# Autodesk Inventor assembly: PowerHub
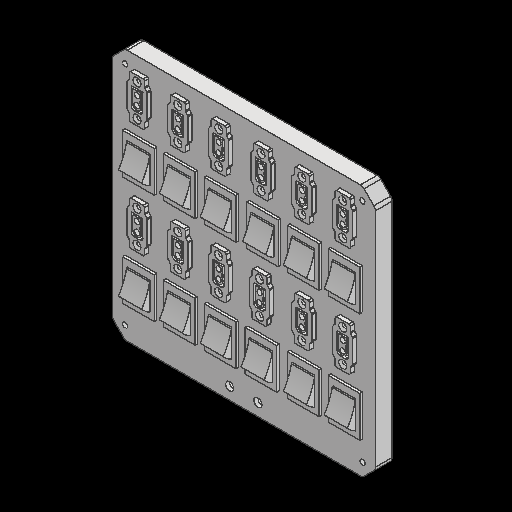
[picture p0: Inventor's stored thumbnail of the model, 512x512]
Saved by Autodesk Inventor 2025.2 (Build 292293000, 293)
## iProperties
Created: 2026-06-06
Part Number: PowerHub
Document SubType Name: Assembly
Designer: valer
Author: valer
## Documents named in this file (4)
- C:\Users\valer\Desktop\str1ker\cad\PowerHub.iam
- C:\Users\valer\Desktop\str1ker\cad\PowerHub.ipt
- C:\Users\valer\Desktop\str1ker\cad\external\XT60E-F.ipt
- C:\Users\valer\Desktop\str1ker\cad\external\IlluminatedSwitch12V10A.ipt
## Components (25 placed, 3 different names)
1. PowerHub:1 — Flush:2, Flush:3, Mate:1, Mate:2, Mate:3, Flush:5, Flush:6, Mate:16, Mate:17, Mate:18, Mate:19, Mate:20, Mate:21, Flush:35, Mate:22, Mate:23, Mate:24, Mate:26, Mate:27, Mate:32, Mate:33, Mate:34, Mate:36, Mate:37, Mate:39, Mate:40, Mate:42, Mate:43, Mate:44, Mate:45
2. XT60E-F:1 — Mate:2, Flush:4, Flush:5, Mate:4, Flush:6, Flush:30, Flush:36, Mate:28
3. IlluminatedSwitch12V10A:1 — Mate:3, Flush:4, Mate:4, Mate:25
4. XT60E-F:2 — Mate:16, Flush:30, Flush:31, Mate:28, Mate:29
5. IlluminatedSwitch12V10A:2 — Mate:17
6. XT60E-F:3 — Flush:31, Flush:32, Mate:22, Mate:29
7. IlluminatedSwitch12V10A:3 — Mate:18
8. XT60E-F:4 — Mate:19, Flush:32, Flush:33, Mate:31
9. IlluminatedSwitch12V10A:4 — Mate:34
10. XT60E-F:5 — Mate:20, Flush:33, Flush:34, Mate:30, Mate:31, Flush:43
11. IlluminatedSwitch12V10A:5 — Mate:33
12. XT60E-F:6 — Mate:21, Flush:34, Flush:35, Mate:30, Flush:42
13. IlluminatedSwitch12V10A:6 — Mate:32
14. XT60E-F:7 — Mate:23, Flush:36, Mate:25, Mate:35, Flush:37
15. IlluminatedSwitch12V10A:7 — Mate:24
16. XT60E-F:8 — Mate:26, Mate:35, Flush:37, Flush:38, Mate:38
17. IlluminatedSwitch12V10A:8 — Mate:27
18. XT60E-F:9 — Mate:36, Flush:38, Mate:38, Mate:41, Flush:39
19. IlluminatedSwitch12V10A:9 — Mate:37
20. XT60E-F:10 — Mate:39, Mate:41, Flush:39, Flush:40
21. IlluminatedSwitch12V10A:10 — Mate:40
22. XT60E-F:11 — Flush:40, Flush:41, Flush:43, Mate:42
23. IlluminatedSwitch12V10A:11 — Mate:43
24. XT60E-F:12 — Flush:41, Flush:42, Mate:44
25. IlluminatedSwitch12V10A:12 — Mate:45
## Relationships (75: Mate 45, Flush 30)
- Flush:2: PowerHub:1
- Flush:3: PowerHub:1
- Mate:1: PowerHub:1
- Mate:2: PowerHub:1 ↔ XT60E-F:1
- Mate:3: PowerHub:1 ↔ IlluminatedSwitch12V10A:1
- Flush:4: XT60E-F:1 ↔ IlluminatedSwitch12V10A:1
- Flush:5 (-14.5 mm): PowerHub:1 ↔ XT60E-F:1
- Mate:4 (9.75 mm): XT60E-F:1 ↔ IlluminatedSwitch12V10A:1
- Flush:6 (-10 mm): PowerHub:1 ↔ XT60E-F:1
- [Flush]: XT60E-F:2 ↔ IlluminatedSwitch12V10A:2
- [Mate] (9.75 mm): XT60E-F:2 ↔ IlluminatedSwitch12V10A:2
- [Flush]: XT60E-F:3 ↔ IlluminatedSwitch12V10A:3
- [Mate] (9.75 mm): XT60E-F:3 ↔ IlluminatedSwitch12V10A:3
- [Flush]: XT60E-F:4 ↔ IlluminatedSwitch12V10A:4
- [Mate] (9.75 mm): XT60E-F:4 ↔ IlluminatedSwitch12V10A:4
- [Flush]: XT60E-F:5 ↔ IlluminatedSwitch12V10A:5
- [Mate] (9.75 mm): XT60E-F:5 ↔ IlluminatedSwitch12V10A:5
- [Flush]: XT60E-F:6 ↔ IlluminatedSwitch12V10A:6
- [Mate] (9.75 mm): XT60E-F:6 ↔ IlluminatedSwitch12V10A:6
- [Flush]: XT60E-F:7 ↔ IlluminatedSwitch12V10A:7
- [Mate] (9.75 mm): XT60E-F:7 ↔ IlluminatedSwitch12V10A:7
- [Flush]: XT60E-F:8 ↔ IlluminatedSwitch12V10A:8
- [Mate] (9.75 mm): XT60E-F:8 ↔ IlluminatedSwitch12V10A:8
- [Flush]: XT60E-F:9 ↔ IlluminatedSwitch12V10A:9
- [Mate] (9.75 mm): XT60E-F:9 ↔ IlluminatedSwitch12V10A:9
- [Flush]: XT60E-F:10 ↔ IlluminatedSwitch12V10A:10
- [Mate] (9.75 mm): XT60E-F:10 ↔ IlluminatedSwitch12V10A:10
- [Flush]: XT60E-F:11 ↔ IlluminatedSwitch12V10A:11
- [Mate] (9.75 mm): XT60E-F:11 ↔ IlluminatedSwitch12V10A:11
- [Flush]: XT60E-F:12 ↔ IlluminatedSwitch12V10A:12
- [Mate] (9.75 mm): XT60E-F:12 ↔ IlluminatedSwitch12V10A:12
- Mate:16: PowerHub:1 ↔ XT60E-F:2
- Flush:30: XT60E-F:1 ↔ XT60E-F:2
- Mate:17: PowerHub:1 ↔ IlluminatedSwitch12V10A:2
- Mate:18: PowerHub:1 ↔ IlluminatedSwitch12V10A:3
- Mate:19: PowerHub:1 ↔ XT60E-F:4
- Flush:31: XT60E-F:2 ↔ XT60E-F:3
- Flush:32: XT60E-F:3 ↔ XT60E-F:4
- Mate:20: PowerHub:1 ↔ XT60E-F:5
- Flush:33: XT60E-F:4 ↔ XT60E-F:5
- Mate:21: PowerHub:1 ↔ XT60E-F:6
- Flush:34: XT60E-F:5 ↔ XT60E-F:6
- Flush:35 (14.5 mm): PowerHub:1 ↔ XT60E-F:6
- Mate:22: PowerHub:1 ↔ XT60E-F:3
- Mate:23: PowerHub:1 ↔ XT60E-F:7
- Mate:24: PowerHub:1 ↔ IlluminatedSwitch12V10A:7
- Flush:36: XT60E-F:1 ↔ XT60E-F:7
- Mate:25 (10 mm): IlluminatedSwitch12V10A:1 ↔ XT60E-F:7
- Mate:26: PowerHub:1 ↔ XT60E-F:8
- Mate:27: PowerHub:1 ↔ IlluminatedSwitch12V10A:8
- Mate:28 (16 mm): XT60E-F:1 ↔ XT60E-F:2
- Mate:29 (16 mm): XT60E-F:2 ↔ XT60E-F:3
- Mate:30 (16 mm): XT60E-F:5 ↔ XT60E-F:6
- Mate:31 (16 mm): XT60E-F:4 ↔ XT60E-F:5
- Mate:32: PowerHub:1 ↔ IlluminatedSwitch12V10A:6
- Mate:33: PowerHub:1 ↔ IlluminatedSwitch12V10A:5
- Mate:34: PowerHub:1 ↔ IlluminatedSwitch12V10A:4
- Mate:35 (16 mm): XT60E-F:7 ↔ XT60E-F:8
- Flush:37: XT60E-F:7 ↔ XT60E-F:8
- Mate:36: PowerHub:1 ↔ XT60E-F:9
- Flush:38: XT60E-F:8 ↔ XT60E-F:9
- Mate:37: PowerHub:1 ↔ IlluminatedSwitch12V10A:9
- Mate:38 (16 mm): XT60E-F:8 ↔ XT60E-F:9
- Mate:39: PowerHub:1 ↔ XT60E-F:10
- Mate:40: PowerHub:1 ↔ IlluminatedSwitch12V10A:10
- Mate:41 (16 mm): XT60E-F:9 ↔ XT60E-F:10
- Flush:39: XT60E-F:9 ↔ XT60E-F:10
- Flush:40: XT60E-F:10 ↔ XT60E-F:11
- Flush:41: XT60E-F:11 ↔ XT60E-F:12
- Flush:42: XT60E-F:6 ↔ XT60E-F:12
- Flush:43: XT60E-F:5 ↔ XT60E-F:11
- Mate:42: PowerHub:1 ↔ XT60E-F:11
- Mate:43: PowerHub:1 ↔ IlluminatedSwitch12V10A:11
- Mate:44: PowerHub:1 ↔ XT60E-F:12
- Mate:45: PowerHub:1 ↔ IlluminatedSwitch12V10A:12
## Named parameters: d10_d5 = 0 mm, d11_d7 = 9.75 mm, d13_d5 = 0 mm, d14_d7 = 9.75 mm, d16_d5 = 0 mm, d17_d7 = 9.75 mm, d19_d5 = 0 mm, d20_d7 = 9.75 mm, d22_d5 = 0 mm, d23_d7 = 9.75 mm, d25_d5 = 0 mm, d26_d7 = 9.75 mm, d28_d5 = 0 mm, d29_d7 = 9.75 mm, d31_d5 = 0 mm, d32_d7 = 9.75 mm, d34_d5 = 0 mm, d35_d7 = 9.75 mm, d37_d5 = 0 mm, d38_d7 = 9.75 mm, d40_d5 = 0 mm, d41_d7 = 9.75 mm
